# Autodesk Inventor assembly: EL2-C-100
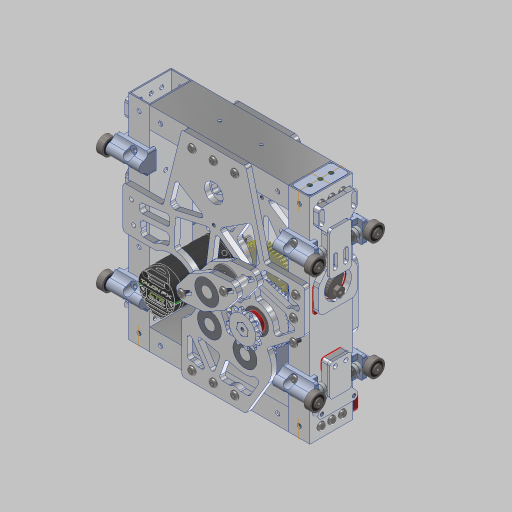
[picture p0: Inventor's stored thumbnail of the model, 512x512]
Saved by Autodesk Inventor 2023.5 (Build 275446000, 446)
## iProperties
Created: 2025-01-11
Part Number: EL2-C-100
Document SubType Name: Assembly
Designer: brand
Mass: 3108.26 g
Surface Area: 6537.92 cm^2
Volume: 1007.04 cm^3
Author: brand
## Documents named in this file (17)
- C:\Users\slick\OneDrive\Desktop\2025-ReefScape---CAD\Elevator\EL2\EL2-C-100.iam
- C:\Users\slick\OneDrive\Desktop\2025-ReefScape---CAD\Elevator\EL2\EL2-C-001.ipt
- C:\Users\slick\OneDrive\Desktop\2025-ReefScape---CAD\Elevator\EL2\EL2-005.ipt
- C:\Users\slick\OneDrive\Desktop\2025-ReefScape---CAD\Elevator\EL2\EL2-C-005.ipt
- C:\Users\slick\OneDrive\Desktop\2025-ReefScape---CAD\COMMON PARTS\WCP Elevator parts\WCP-0323\WCP-0323.iam
- C:\Users\slick\OneDrive\Desktop\2025-ReefScape---CAD\Elevator\EL2-CGB\EL2-CGB-100.iam
- C:\Users\slick\OneDrive\Desktop\2025-ReefScape---CAD\COMMON PARTS\WCP\WCP-0882.ipt
- C:\Users\slick\OneDrive\Desktop\2025-ReefScape---CAD\STEP files\sen36005_3d_model\sen36005_3d_model.iam
- C:\Users\slick\OneDrive\Desktop\2025-ReefScape---CAD\Content Center\en-US\U UNC 2605\Unbrako - 10 x 1 - 32(10).ipt
- C:\Users\slick\OneDrive\Desktop\2025-ReefScape---CAD\Content Center\en-US\U UNC 2605\Unbrako - 10 x 3_8 - 32(10).ipt
- C:\Users\slick\OneDrive\Desktop\2025-ReefScape---CAD\Elevator\EL2\EL2-C-200.iam
- C:\Users\slick\OneDrive\Desktop\2025-ReefScape---CAD\Elevator\EL2\EL2-C-300.iam
- C:\Users\slick\OneDrive\Desktop\2025-ReefScape---CAD\Elevator\EL2\EL2-C-006.ipt
- C:\Users\slick\OneDrive\Desktop\2025-ReefScape---CAD\Elevator\EL2\EL2-019.ipt
- C:\Users\slick\OneDrive\Desktop\2025-ReefScape---CAD\Elevator\Homing Sensor\HS-002.ipt
- C:\Users\slick\OneDrive\Desktop\2025-ReefScape---CAD\Elevator\EL2\EL2-040.ipt
- C:\Users\slick\OneDrive\Desktop\2025-ReefScape---CAD\COMMON PARTS\E2_150_40_1PZ_1\E2_150_40_1PZ_1.iam
## Components (65 placed, 16 different names)
1. EL2-C-001:1 — Flush:4, Flush:8, Mate:10, Flush:9, Flush:11, Symmetry:2, Insert:76, Insert:77, Insert:145, Insert:147, Insert:150
2. EL2-C-005:2 — Insert:2, Angle:2, Flush:4, Mate:10, Insert:15, Insert:18, Insert:21, Insert:25, Insert:26, Insert:27, Mate:11, Symmetry:1, Insert:45, Insert:46, Insert:47, Insert:48, Insert:75, Insert:79, Insert:82, Insert:83, Flush:74, Insert:140, Insert:141, Insert:142, Insert:143, Insert:146, Insert:151
3. EL2-C-005:1 — Insert:8, Insert:10, Insert:32, Insert:33, Mate:12, Flush:12, Insert:34, Insert:37, Insert:38, Insert:39, Insert:40, Insert:41, Symmetry:1, Insert:49, Insert:50, Insert:74, Insert:84, Insert:85, Insert:86, Insert:87, Insert:88, Insert:89, Insert:132, Insert:133, Insert:138, Insert:139, Insert:144
4. EL2-C-001:4 — Flush:10, Flush:11, Mate:11, Mate:12, Flush:12, Symmetry:2, Insert:51, Insert:52, Angle:3
5. EL2-005:1 — Insert:2, Angle:2, Flush:9
6. EL2-005:2 — Insert:8, Flush:8
7. EL2-005:3 — Insert:10, Flush:10, Insert:32, Insert:33
8. WCP-0323:1 [sub-assembly] — Insert:34, Insert:49, Insert:100
9. WCP-0323:2 [sub-assembly] — Insert:40, Insert:41
10. WCP-0323:3 [sub-assembly] — Insert:38, Insert:39, Insert:131
11. WCP-0323:4 [sub-assembly] — Insert:25, Insert:27, Insert:46, Insert:98
12. WCP-0323:5 [sub-assembly] — Insert:18, Insert:26, Insert:130
13. WCP-0323:6 [sub-assembly] — Insert:15, Insert:48, Insert:102
14. WCP-0323:7 [sub-assembly] — Insert:21, Insert:45, Insert:47, Insert:99
15. WCP-0323:8 [sub-assembly] — Insert:37, Insert:50, Insert:101
16. EL2-CGB-100:1 [sub-assembly] — Insert:51, Insert:52, Mate:48, Mate:49, Mate:52, Mate:53, Mate:54, Mate:55, Mate:56, Mate:57, Mate:58, Mate:59, Mate:60, Mate:61, Mate:62, Mate:63, Mate:66, Mate:67, Mate:68, Mate:69, Insert:103, Insert:105, Insert:106, Insert:115, Insert:116, Insert:117, Insert:118, Insert:120, Insert:121, Insert:123, Insert:124, Insert:125, Insert:126, Insert:129
17. WCP-0882:1 — Insert:75
18. WCP-0882:2 — Insert:74
19. sen36005_3d_model:1 [sub-assembly] — Insert:76, Insert:77
20. Unbrako UNC Hex Socket Button Cap - Inch 10 x 1:14 — Mate:48, Mate:49
21. Unbrako UNC Hex Socket Button Cap - Inch 10 x 1:16 — Mate:52, Mate:53
22. Unbrako UNC Hex Socket Button Cap - Inch 10 x 1:17 — Mate:54, Mate:55
23. Unbrako UNC Hex Socket Button Cap - Inch 10 x 1:18 — Mate:56, Mate:57
24. Unbrako UNC Hex Socket Button Cap - Inch 10 x 1:19 — Mate:58, Mate:59
25. Unbrako UNC Hex Socket Button Cap - Inch 10 x 1:20 — Mate:60, Mate:61
26. Unbrako UNC Hex Socket Button Cap - Inch 10 x 1:21 — Mate:62, Mate:63
27. Unbrako UNC Hex Socket Button Cap - Inch 10 x 1:23 — Mate:66, Mate:67
28. Unbrako UNC Hex Socket Button Cap - Inch 10 x 1:24 — Mate:68, Mate:69
29. Unbrako UNC Hex Socket Button Cap - Inch 10 x 3/8:2 — Insert:79
30. Unbrako UNC Hex Socket Button Cap - Inch 10 x 3/8:5 — Insert:82
31. Unbrako UNC Hex Socket Button Cap - Inch 10 x 3/8:6 — Insert:83
32. Unbrako UNC Hex Socket Button Cap - Inch 10 x 3/8:7 — Insert:84
33. Unbrako UNC Hex Socket Button Cap - Inch 10 x 3/8:8 — Insert:85
34. Unbrako UNC Hex Socket Button Cap - Inch 10 x 3/8:9 — Insert:86
35. Unbrako UNC Hex Socket Button Cap - Inch 10 x 3/8:10 — Insert:87
36. Unbrako UNC Hex Socket Button Cap - Inch 10 x 3/8:11 — Insert:88
37. Unbrako UNC Hex Socket Button Cap - Inch 10 x 3/8:12 — Insert:89
38. Unbrako UNC Hex Socket Button Cap - Inch 10 x 1:33 — Insert:98
39. Unbrako UNC Hex Socket Button Cap - Inch 10 x 1:34 — Insert:99
40. Unbrako UNC Hex Socket Button Cap - Inch 10 x 1:35 — Insert:100
41. Unbrako UNC Hex Socket Button Cap - Inch 10 x 1:36 — Insert:101
42. Unbrako UNC Hex Socket Button Cap - Inch 10 x 1:37 — Insert:102
43. Unbrako UNC Hex Socket Button Cap - Inch 10 x 3/8:13 — Insert:103
44. Unbrako UNC Hex Socket Button Cap - Inch 10 x 3/8:15 — Insert:105
45. Unbrako UNC Hex Socket Button Cap - Inch 10 x 3/8:16 — Insert:106
46. Unbrako UNC Hex Socket Button Cap - Inch 10 x 1:42 — Insert:115
47. Unbrako UNC Hex Socket Button Cap - Inch 10 x 1:43 — Insert:116
48. Unbrako UNC Hex Socket Button Cap - Inch 10 x 1:44 — Insert:117
49. Unbrako UNC Hex Socket Button Cap - Inch 10 x 1:45 — Insert:118
50. Unbrako UNC Hex Socket Button Cap - Inch 10 x 1:47 — Insert:120
51. Unbrako UNC Hex Socket Button Cap - Inch 10 x 1:48 — Insert:121
52. Unbrako UNC Hex Socket Button Cap - Inch 10 x 1:50 — Insert:123
53. Unbrako UNC Hex Socket Button Cap - Inch 10 x 1:51 — Insert:124
54. Unbrako UNC Hex Socket Button Cap - Inch 10 x 1:52 — Insert:125
55. Unbrako UNC Hex Socket Button Cap - Inch 10 x 1:53 — Insert:126
56. Unbrako UNC Hex Socket Button Cap - Inch 10 x 1:56 — Insert:129
57. Unbrako UNC Hex Socket Button Cap - Inch 10 x 1:57 — Insert:130
58. Unbrako UNC Hex Socket Button Cap - Inch 10 x 1:58 — Insert:131
59. EL2-C-200:1 [sub-assembly] — Insert:132, Insert:133
60. EL2-C-300:2 [sub-assembly] — Insert:138, Insert:139
61. EL2-C-006:1 — Angle:3, Flush:74, Insert:140, Insert:141
62. EL2-019:1 — Insert:142, Insert:143
63. HS-002:1 — Insert:144, Insert:145
64. EL2-040:1 — Insert:146, Insert:147, Insert:150, Insert:151, Insert:152, Insert:153
65. E2_150_40_1PZ_1:1 [sub-assembly] — Insert:152, Insert:153
## Relationships (109: Insert 75, Mate 23, Flush 7, Angle 2, Symmetry 2)
- Insert:2: EL2-C-005:2 ↔ EL2-005:1
- Angle:2 (0 deg): EL2-C-005:2 ↔ EL2-005:1
- Insert:8: EL2-C-005:1 ↔ EL2-005:2
- Insert:10: EL2-C-005:1 ↔ EL2-005:3
- Flush:4: EL2-C-001:1 ↔ EL2-C-005:2
- Flush:8: EL2-C-001:1 ↔ EL2-005:2
- Mate:10: EL2-C-001:1 ↔ EL2-C-005:2
- Flush:9: EL2-C-001:1 ↔ EL2-005:1
- Flush:10: EL2-C-001:4 ↔ EL2-005:3
- Flush:11: EL2-C-001:1 ↔ EL2-C-001:4
- Insert:15: EL2-C-005:2 ↔ WCP-0323:6
- Insert:18: EL2-C-005:2 ↔ WCP-0323:5
- Insert:21: EL2-C-005:2 ↔ WCP-0323:7
- Insert:25: EL2-C-005:2 ↔ WCP-0323:4
- Insert:26: EL2-C-005:2 ↔ WCP-0323:5
- Insert:27: EL2-C-005:2 ↔ WCP-0323:4
- Insert:32: EL2-C-005:1 ↔ EL2-005:3
- Insert:33: EL2-C-005:1 ↔ EL2-005:3
- Mate:11: EL2-C-005:2 ↔ EL2-C-001:4
- Mate:12: EL2-C-005:1 ↔ EL2-C-001:4
- Flush:12: EL2-C-005:1 ↔ EL2-C-001:4
- Insert:34: EL2-C-005:1 ↔ WCP-0323:1
- Insert:37: EL2-C-005:1 ↔ WCP-0323:8
- Insert:38: EL2-C-005:1 ↔ WCP-0323:3
- Insert:39: EL2-C-005:1 ↔ WCP-0323:3
- Insert:40: EL2-C-005:1 ↔ WCP-0323:2
- Insert:41: EL2-C-005:1 ↔ WCP-0323:2
- Symmetry:1: EL2-C-005:2 ↔ EL2-C-005:1
- Symmetry:2: EL2-C-001:1 ↔ EL2-C-001:4
- Mate:13
- Mate:14
- Insert:45: EL2-C-005:2 ↔ WCP-0323:7
- Insert:46: EL2-C-005:2 ↔ WCP-0323:4
- Insert:47: EL2-C-005:2 ↔ WCP-0323:7
- Insert:48: EL2-C-005:2 ↔ WCP-0323:6
- Insert:49: EL2-C-005:1 ↔ WCP-0323:1
- Insert:50: EL2-C-005:1 ↔ WCP-0323:8
- Insert:51: EL2-C-001:4 ↔ EL2-CGB-100:1
- Insert:52: EL2-C-001:4 ↔ EL2-CGB-100:1
- Insert:74: EL2-C-005:1 ↔ WCP-0882:2
- Insert:75: EL2-C-005:2 ↔ WCP-0882:1
- Insert:76: EL2-C-001:1 ↔ sen36005_3d_model:1
- Insert:77: EL2-C-001:1 ↔ sen36005_3d_model:1
- Mate:48: EL2-CGB-100:1 ↔ Unbrako UNC Hex Socket Button Cap - Inch 10 x 1:14
- Mate:49: EL2-CGB-100:1 ↔ Unbrako UNC Hex Socket Button Cap - Inch 10 x 1:14
- Mate:52: EL2-CGB-100:1 ↔ Unbrako UNC Hex Socket Button Cap - Inch 10 x 1:16
- Mate:53: EL2-CGB-100:1 ↔ Unbrako UNC Hex Socket Button Cap - Inch 10 x 1:16
- Mate:54: EL2-CGB-100:1 ↔ Unbrako UNC Hex Socket Button Cap - Inch 10 x 1:17
- Mate:55: EL2-CGB-100:1 ↔ Unbrako UNC Hex Socket Button Cap - Inch 10 x 1:17
- Mate:56: EL2-CGB-100:1 ↔ Unbrako UNC Hex Socket Button Cap - Inch 10 x 1:18
- Mate:57: EL2-CGB-100:1 ↔ Unbrako UNC Hex Socket Button Cap - Inch 10 x 1:18
- Mate:58: EL2-CGB-100:1 ↔ Unbrako UNC Hex Socket Button Cap - Inch 10 x 1:19
- Mate:59: EL2-CGB-100:1 ↔ Unbrako UNC Hex Socket Button Cap - Inch 10 x 1:19
- Mate:60: EL2-CGB-100:1 ↔ Unbrako UNC Hex Socket Button Cap - Inch 10 x 1:20
- Mate:61: EL2-CGB-100:1 ↔ Unbrako UNC Hex Socket Button Cap - Inch 10 x 1:20
- Mate:62: EL2-CGB-100:1 ↔ Unbrako UNC Hex Socket Button Cap - Inch 10 x 1:21
- Mate:63: EL2-CGB-100:1 ↔ Unbrako UNC Hex Socket Button Cap - Inch 10 x 1:21
- Mate:66: EL2-CGB-100:1 ↔ Unbrako UNC Hex Socket Button Cap - Inch 10 x 1:23
- Mate:67: EL2-CGB-100:1 ↔ Unbrako UNC Hex Socket Button Cap - Inch 10 x 1:23
- Mate:68: EL2-CGB-100:1 ↔ Unbrako UNC Hex Socket Button Cap - Inch 10 x 1:24
- Mate:69: EL2-CGB-100:1 ↔ Unbrako UNC Hex Socket Button Cap - Inch 10 x 1:24
- Insert:79: EL2-C-005:2 ↔ Unbrako UNC Hex Socket Button Cap - Inch 10 x 3/8:2
- Insert:82: EL2-C-005:2 ↔ Unbrako UNC Hex Socket Button Cap - Inch 10 x 3/8:5
- Insert:83: EL2-C-005:2 ↔ Unbrako UNC Hex Socket Button Cap - Inch 10 x 3/8:6
- Insert:84: EL2-C-005:1 ↔ Unbrako UNC Hex Socket Button Cap - Inch 10 x 3/8:7
- Insert:85: EL2-C-005:1 ↔ Unbrako UNC Hex Socket Button Cap - Inch 10 x 3/8:8
- Insert:86: EL2-C-005:1 ↔ Unbrako UNC Hex Socket Button Cap - Inch 10 x 3/8:9
- Insert:87: EL2-C-005:1 ↔ Unbrako UNC Hex Socket Button Cap - Inch 10 x 3/8:10
- Insert:88: EL2-C-005:1 ↔ Unbrako UNC Hex Socket Button Cap - Inch 10 x 3/8:11
- Insert:89: EL2-C-005:1 ↔ Unbrako UNC Hex Socket Button Cap - Inch 10 x 3/8:12
- Insert:98: WCP-0323:4 ↔ Unbrako UNC Hex Socket Button Cap - Inch 10 x 1:33
- Insert:99: WCP-0323:7 ↔ Unbrako UNC Hex Socket Button Cap - Inch 10 x 1:34
- Insert:100: WCP-0323:1 ↔ Unbrako UNC Hex Socket Button Cap - Inch 10 x 1:35
- Insert:101: WCP-0323:8 ↔ Unbrako UNC Hex Socket Button Cap - Inch 10 x 1:36
- Insert:102: WCP-0323:6 ↔ Unbrako UNC Hex Socket Button Cap - Inch 10 x 1:37
- Insert:103: EL2-CGB-100:1 ↔ Unbrako UNC Hex Socket Button Cap - Inch 10 x 3/8:13
- Insert:105: EL2-CGB-100:1 ↔ Unbrako UNC Hex Socket Button Cap - Inch 10 x 3/8:15
- Insert:106: EL2-CGB-100:1 ↔ Unbrako UNC Hex Socket Button Cap - Inch 10 x 3/8:16
- Insert:115: EL2-CGB-100:1 ↔ Unbrako UNC Hex Socket Button Cap - Inch 10 x 1:42
- Insert:116: EL2-CGB-100:1 ↔ Unbrako UNC Hex Socket Button Cap - Inch 10 x 1:43
- Insert:117: EL2-CGB-100:1 ↔ Unbrako UNC Hex Socket Button Cap - Inch 10 x 1:44
- Insert:118: EL2-CGB-100:1 ↔ Unbrako UNC Hex Socket Button Cap - Inch 10 x 1:45
- Insert:120: EL2-CGB-100:1 ↔ Unbrako UNC Hex Socket Button Cap - Inch 10 x 1:47
- Insert:121: EL2-CGB-100:1 ↔ Unbrako UNC Hex Socket Button Cap - Inch 10 x 1:48
- Insert:123: EL2-CGB-100:1 ↔ Unbrako UNC Hex Socket Button Cap - Inch 10 x 1:50
- Insert:124: EL2-CGB-100:1 ↔ Unbrako UNC Hex Socket Button Cap - Inch 10 x 1:51
- Insert:125: EL2-CGB-100:1 ↔ Unbrako UNC Hex Socket Button Cap - Inch 10 x 1:52
- Insert:126: EL2-CGB-100:1 ↔ Unbrako UNC Hex Socket Button Cap - Inch 10 x 1:53
- Insert:129: EL2-CGB-100:1 ↔ Unbrako UNC Hex Socket Button Cap - Inch 10 x 1:56
- Insert:130: WCP-0323:5 ↔ Unbrako UNC Hex Socket Button Cap - Inch 10 x 1:57
- Insert:131: WCP-0323:3 ↔ Unbrako UNC Hex Socket Button Cap - Inch 10 x 1:58
- Insert:132: EL2-C-005:1 ↔ EL2-C-200:1
- Insert:133: EL2-C-005:1 ↔ EL2-C-200:1
- Insert:138: EL2-C-005:1 ↔ EL2-C-300:2
- Insert:139: EL2-C-005:1 ↔ EL2-C-300:2
- Angle:3 (0 deg): EL2-C-001:4 ↔ EL2-C-006:1
- Flush:74: EL2-C-005:2 ↔ EL2-C-006:1
- Insert:140: EL2-C-005:2 ↔ EL2-C-006:1
- Insert:141: EL2-C-005:2 ↔ EL2-C-006:1
- Insert:142: EL2-C-005:2 ↔ EL2-019:1
- Insert:143: EL2-C-005:2 ↔ EL2-019:1
- Insert:144: EL2-C-005:1 ↔ HS-002:1
- Insert:145: EL2-C-001:1 ↔ HS-002:1
- Insert:146: EL2-C-005:2 ↔ EL2-040:1
- Insert:147: EL2-C-001:1 ↔ EL2-040:1
- Insert:150: EL2-C-001:1 ↔ EL2-040:1
- Insert:151: EL2-C-005:2 ↔ EL2-040:1
- Insert:152: EL2-040:1 ↔ E2_150_40_1PZ_1:1
- Insert:153: EL2-040:1 ↔ E2_150_40_1PZ_1:1
